# Autodesk Inventor assembly: 5 Barras Simplificado
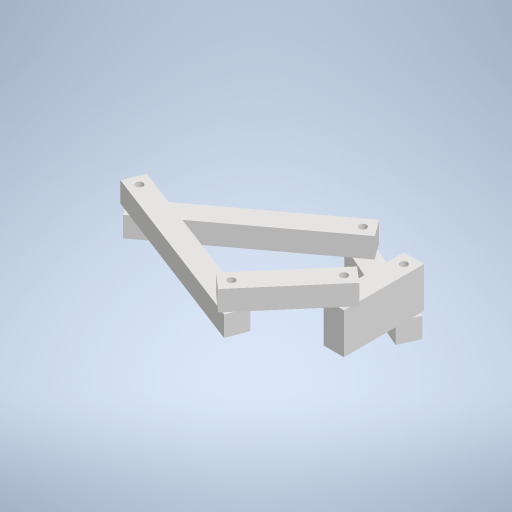
[picture p0: Inventor's stored thumbnail of the model, 512x512]
Saved by Autodesk Inventor 2024.2 (Build 282272000, 272)
## iProperties
Created: 2024-02-01
Part Number: 5 Barras Simplificado
Document SubType Name: Assembly
Designer: juanp
Author: juanp
## Documents named in this file (6)
- C:\Users\jp.reyesf\OneDrive - Universidad de los andes\Uniandes\Tesis Maestria\CAD\5 Barras Simplificado.iam
- C:\Users\jp.reyesf\OneDrive - Universidad de los andes\Uniandes\Tesis Maestria\CAD\Solid1.ipt
- C:\Users\jp.reyesf\OneDrive - Universidad de los andes\Uniandes\Tesis Maestria\CAD\Solid2.ipt
- C:\Users\jp.reyesf\OneDrive - Universidad de los andes\Uniandes\Tesis Maestria\CAD\Solid3.ipt
- C:\Users\jp.reyesf\OneDrive - Universidad de los andes\Uniandes\Tesis Maestria\CAD\Solid4.ipt
- C:\Users\jp.reyesf\OneDrive - Universidad de los andes\Uniandes\Tesis Maestria\CAD\Solid5.ipt
## Components (5 placed, 5 different names)
1. Solid1:1 — Mate:4, Mate:5, Mate:9, Mate:10
2. Solid2:1 — Mate:3, Mate:4, Mate:8, Mate:9
3. Solid3:1 — Mate:2, Mate:3, Mate:7, Mate:8
4. Solid4:1 — Mate:1, Mate:2, Mate:6, Mate:7
5. Solid5:1 — Mate:1, Mate:5, Mate:6, Mate:10
## Relationships (10: Mate 10)
- Mate:1: Solid4:1 ↔ Solid5:1
- Mate:2: Solid3:1 ↔ Solid4:1
- Mate:3: Solid2:1 ↔ Solid3:1
- Mate:4: Solid1:1 ↔ Solid2:1
- Mate:5: Solid1:1 ↔ Solid5:1
- Mate:6: Solid4:1 ↔ Solid5:1
- Mate:7: Solid3:1 ↔ Solid4:1
- Mate:8: Solid2:1 ↔ Solid3:1
- Mate:9: Solid1:1 ↔ Solid2:1
- Mate:10: Solid1:1 ↔ Solid5:1
